# Autodesk Inventor assembly: robotic_arm
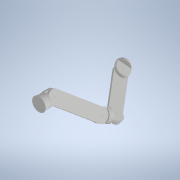
[picture p0: Inventor's stored thumbnail of the model, 180x180]
Saved by Autodesk Inventor 2022 (Build 260153000, 153)
## iProperties
Created: 2022-02-25
Part Number: robotic_arm
Document SubType Name: Assembly
Designer: Dan
Author: Dan
## Documents named in this file (5)
- C:\Users\Dan\Documents\uni\Extracurricular\OWR\2022\ros-packages\robotic_arm_cad\robotic_arm.iam
- C:\Users\Dan\Documents\uni\Extracurricular\OWR\2022\ros-packages\robotic_arm_cad\shoulder_base.ipt
- C:\Users\Dan\Documents\uni\Extracurricular\OWR\2022\ros-packages\robotic_arm_cad\joint_hub.ipt
- joint_hub.ipt
- C:\Users\Dan\Documents\uni\Extracurricular\OWR\2022\ros-packages\robotic_arm_cad\arm_link.ipt
## Components (7 placed, 3 different names)
1. shoulder_base:1 — Rotational:1
2. joint_hub:1 — Rotational:1, Rotational:2
3. arm_link:1 — Rotational:2, Rotational:3
4. joint_hub:2 — Rotational:3, Rotational:4
5. joint_hub:3 — Rotational:4, Rotational:5
6. arm_link:2 — Rotational:5, Rotational:6
7. joint_hub:4 — Rotational:6
## Relationships (6: RevoluteJoint 6)
- Rotational:1 [RevoluteJoint]: shoulder_base:1 ↔ joint_hub:1
- Rotational:2 [RevoluteJoint]: joint_hub:1 ↔ arm_link:1
- Rotational:3 [RevoluteJoint]: arm_link:1 ↔ joint_hub:2
- Rotational:4 [RevoluteJoint]: joint_hub:2 ↔ joint_hub:3
- Rotational:5 [RevoluteJoint]: joint_hub:3 ↔ arm_link:2
- Rotational:6 [RevoluteJoint]: arm_link:2 ↔ joint_hub:4
